# Autodesk Inventor assembly: Clutch Concept
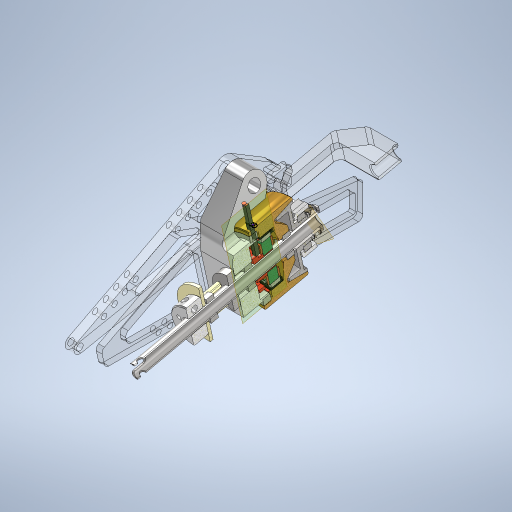
[picture p0: Inventor's stored thumbnail of the model, 512x512]
Saved by Autodesk Inventor 2023.4 (Build 274418000, 418)
## iProperties
Created: 2024-02-03
Part Number: Clutch Concept
Document SubType Name: Assembly
Designer: Nathan Cai
Mass: 481.212 g
Surface Area: 1239.13 cm^2
Volume: 142.768 cm^3
Density: 3.37059 g/cm^3
Author: Nathan Cai
## Documents named in this file (17)
- E:\Documents\Inventor\Bleep V1.5\Clutch Concept.iam
- E:\Documents\Inventor\Bleep V1.5\Flywheel.ipt
- E:\Documents\Inventor\Bleep V1.5\Thrust Bearing.ipt
- E:\Documents\Inventor\Bleep V1.5\BB 13x19x4.ipt
- E:\Documents\Inventor\Bleep V1.5\Cup.ipt
- E:\Documents\Inventor\Bleep V1.5\1561T741_Stacked Wave Disc Spring\1561T741_Stacked Wave Disc Spring.ipt
- E:\Documents\Inventor\Bleep V1.5\AKK RS2205 2300KV\AKK RS2205 2300KV.iam
- E:\Documents\Inventor\Bleep V1.5\BB 37mm x 30mm x 4mm.ipt
- E:\Documents\Inventor\Bleep V1.5\Motor Plate.ipt
- E:\Documents\Inventor\Bleep V1.5\Uprights.ipt
- E:\Documents\Inventor\Bleep V1.5\5172T23_Metal Gear - 20 Degree Pressure Angle\5172T23_Metal Gear - 20 Degree Pressure Angle.ipt
- E:\Documents\Inventor\Bleep V1.5\BB .25x.5x.1875 - Flangeless.ipt
- E:\Documents\Inventor\Bleep V1.5\Shaft - Flywheel C.ipt
- E:\Documents\Inventor\Bleep V1.5\Clutch C.ipt
- E:\Documents\Inventor\Bleep V1.5\Collar.ipt
- E:\Documents\Inventor\Bleep V1.5\Rack - Slot.ipt
- E:\Documents\Inventor\Bleep V1.5\Spring Spool.ipt
## Components (19 placed, 16 different names)
1. BB .25x.5x.1875 - Flangeless:3 — Mate:470
2. Spring Spool:1 — Mate:476, Mate:478
3. Flywheel:1 — Mate:37, Flush:102, Mate:104, Mate:105, Mate:275, Mate:309, Flush:154
4. Shaft - Flywheel C:1 — Mate:306, Mate:307, Mate:308, Mate:310, Mate:311, Mate:312, Mate:313, Mate:315, Angle:4, Mate:319, Mate:324, Mate:470, Mate:479
5. Clutch C:1 — Mate:308, Angle:4, Flush:154
6. Rack - Slot:1 — Angle:1, Angle:3, Rotation/Translation:1, Mate:315, Mate:313, Mate:479
7. Cup:1 — Mate:26, Mate:27, Angle:1
8. AKK RS2205 2300KV:1 [sub-assembly] — Mate:37, Flush:102, Mate:426
9. Motor Plate:1 — Mate:106, Mate:107, Flush:106, Mate:426, Mate:481, Mate:480, Mate:482, Mate:483, Mate:484, Flush:155
10. 1561T741_Stacked Wave Disc Spring:1 — Mate:311, Mate:312
11. Thrust Bearing:1 — Mate:319, Mate:475
12. Collar:1 — Mate:324, Mate:475, Mate:476, Mate:478
13. Uprights:1 — Flush:103, Flush:104, Mate:138, Mate:480, Mate:484, Flush:155
14. Uprights:2 — Flush:103, Flush:104, Mate:482
15. 5172T23_Metal Gear - 20 Degree Pressure Angle:1 — Mate:138, Angle:3, Rotation/Translation:1, Mate:483
16. BB .25x.5x.1875 - Flangeless:1 — Flush:106, Mate:310
17. BB 13x19x4:1 — Mate:26, Mate:27
18. BB 37mm x 30mm x 4mm:1 — Mate:104, Mate:105, Mate:106, Mate:107
19. BB .25x.5x.1875 - Flangeless:2 — Mate:275, Mate:306, Mate:307, Mate:309
## Relationships (43: Mate 33, Flush 6, Angle 3, RelateRotateTranslate 1)
- [Mate]: Clutch C:1 ↔ BB 13x19x4:1
- [Mate]: Clutch C:1 ↔ BB 13x19x4:1
- Mate:26: Cup:1 ↔ BB 13x19x4:1
- Mate:27: Cup:1 ↔ BB 13x19x4:1
- Mate:37: Flywheel:1 ↔ AKK RS2205 2300KV:1
- Angle:1 (0 deg): Rack - Slot:1 ↔ Cup:1
- Flush:102: Flywheel:1 ↔ AKK RS2205 2300KV:1
- Mate:104: Flywheel:1 ↔ BB 37mm x 30mm x 4mm:1
- Mate:105: Flywheel:1 ↔ BB 37mm x 30mm x 4mm:1
- Mate:106: Motor Plate:1 ↔ BB 37mm x 30mm x 4mm:1
- Mate:107: Motor Plate:1 ↔ BB 37mm x 30mm x 4mm:1
- Flush:103: Uprights:1 ↔ Uprights:2
- Flush:104: Uprights:1 ↔ Uprights:2
- Mate:138: Uprights:1 ↔ 5172T23_Metal Gear - 20 Degree Pressure Angle:1
- Flush:106 (5.1594 mm): Motor Plate:1 ↔ BB .25x.5x.1875 - Flangeless:1
- Angle:3 (0 deg): Rack - Slot:1 ↔ 5172T23_Metal Gear - 20 Degree Pressure Angle:1
- Rotation/Translation:1 [RelateRotateTranslate] (159.5929 mm): Rack - Slot:1 ↔ 5172T23_Metal Gear - 20 Degree Pressure Angle:1
- Mate:315 (31.75 mm): Shaft - Flywheel C:1 ↔ Rack - Slot:1
- Mate:275: Flywheel:1 ↔ BB .25x.5x.1875 - Flangeless:2
- Mate:306: Shaft - Flywheel C:1 ↔ BB .25x.5x.1875 - Flangeless:2
- Mate:307: Shaft - Flywheel C:1 ↔ BB .25x.5x.1875 - Flangeless:2
- Mate:308: Shaft - Flywheel C:1 ↔ Clutch C:1
- Mate:309: Flywheel:1 ↔ BB .25x.5x.1875 - Flangeless:2
- Mate:310: Shaft - Flywheel C:1 ↔ BB .25x.5x.1875 - Flangeless:1
- Mate:311: Shaft - Flywheel C:1 ↔ 1561T741_Stacked Wave Disc Spring:1
- Mate:312: Shaft - Flywheel C:1 ↔ 1561T741_Stacked Wave Disc Spring:1
- Mate:313: Shaft - Flywheel C:1 ↔ Rack - Slot:1
- Angle:4 (0 deg): Shaft - Flywheel C:1 ↔ Clutch C:1
- Mate:319: Shaft - Flywheel C:1 ↔ Thrust Bearing:1
- Mate:324: Shaft - Flywheel C:1 ↔ Collar:1
- Mate:426: AKK RS2205 2300KV:1 ↔ Motor Plate:1
- Mate:470: BB .25x.5x.1875 - Flangeless:3 ↔ Shaft - Flywheel C:1
- Mate:475 (14.2875 mm): Thrust Bearing:1 ↔ Collar:1
- Mate:476: Spring Spool:1 ↔ Collar:1
- Mate:478: Spring Spool:1 ↔ Collar:1
- Mate:481: Motor Plate:1
- Mate:479: Shaft - Flywheel C:1 ↔ Rack - Slot:1
- Flush:154: Flywheel:1 ↔ Clutch C:1
- Mate:480: Motor Plate:1 ↔ Uprights:1
- Mate:482: Motor Plate:1 ↔ Uprights:2
- Mate:483: Motor Plate:1 ↔ 5172T23_Metal Gear - 20 Degree Pressure Angle:1
- Mate:484 (-3.175 mm): Motor Plate:1 ↔ Uprights:1
- Flush:155: Motor Plate:1 ↔ Uprights:1
